# Autodesk Inventor assembly: 3D HUMAN
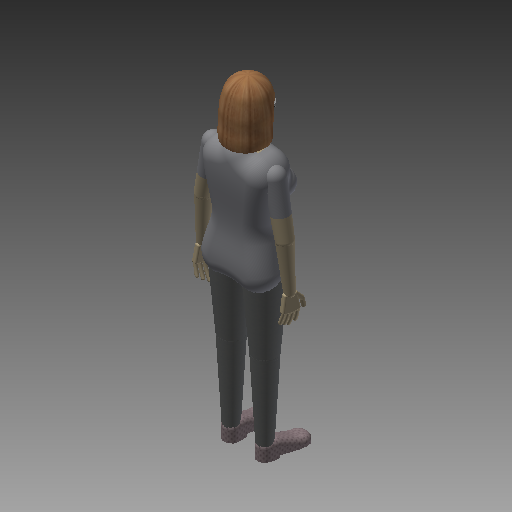
[picture p0: Inventor's stored thumbnail of the model, 512x512]
Saved by Autodesk Inventor 2019 (Build 230136000, 136)
## iProperties
Category: ASSY
Shininess: 64.0
Length Units: 11272
Angle Units: 11279
Time Units: 11290
Mass Units: 11286
Length Display Precision: 3
Angle Display Precision: 2
Compacted: True
Part Number: 3D HUMAN
Document SubType Name: Assembly
Created: 2003-03-22
Designer: M.F.
Catalog Web Link: www.apollocanard.com
Density: 0.0
Volumn: 0.0
Area: 0.0
PropertySet Name: Model Information
Control State: 0
Master: False
Checked Out: False
Title: iMandy
Author: M.F.
## Documents named in this file (14)
- \\Mac\Home\Downloads\iManikins\iMandy\iMandy.iam
- \\Mac\Home\Downloads\iManikins\iMandy\iMandy - 2D BODY.ipt
- \\Mac\Home\Downloads\iManikins\iMandy\iMandy - HAIR.ipt
- \\Mac\Home\Downloads\iManikins\iMandy\iMandy - HEAD.ipt
- \\Mac\Home\Downloads\iManikins\iMandy\iMandy - ARM UPPER.ipt
- \\Mac\Home\Downloads\iManikins\iMandy\iMandy - ARM LOWER.ipt
- \\Mac\Home\Downloads\iManikins\iMandy\iMandy - LEG UPPER.ipt
- \\Mac\Home\Downloads\iManikins\iMandy\iMandy - LEG LOWER.ipt
- \\Mac\Home\Downloads\iManikins\iMandy\iMandy - FOOT.ipt
- \\Mac\Home\Downloads\iManikins\iMandy\iMandy - HAND.ipt
- \\Mac\Home\Downloads\iManikins\iMandy\iMandy - FINGERS LEFT.ipt
- \\Mac\Home\Downloads\iManikins\iMandy\iMandy - FINGERS RIGHT.ipt
- \\Mac\Home\Downloads\iManikins\iMandy\iMandy - SHADES.ipt
- \\Mac\Home\Downloads\iManikins\iMandy\iMandy - TORSO.ipt
## Components (19 placed, 13 different names)
1. iMandy - 2D BODY:1 — Flush:1, Flush:2, Flush:7
2. iMandy - TORSO:1 — Flush:4, Flush:6, LEFT FOOT TWIST ANGLE, LEG STRADDLE DIST1, LEG STRADDLE DIST2, Flush:7, LEFT FOOT FLAT, RIGHT FOOT FLAT, Tangent:3, Mate:17
3. iMandy - ARM UPPER:1 — Mate:1
4. iMandy - ARM LOWER:1 — Mate:1, Mate:4
5. iMandy - LEG UPPER:1 — Mate:2
6. iMandy - LEG LOWER:1 — Mate:2, Mate:3, LEG STRADDLE DIST1, Tangent:1
7. iMandy - FOOT:1 — Mate:3, LEFT FOOT TWIST ANGLE, Tangent:1, LEFT FOOT FLAT
8. iMandy - HAND:1 — Mate:4, Mate:5, Mate:6, LEFT FINGERS CLOSED ANGLE
9. iMandy - FINGERS LEFT:1 — Mate:5, Mate:6, LEFT FINGERS CLOSED ANGLE
10. iMandy - ARM UPPER:2 — Mate:7
11. iMandy - ARM LOWER:2 — Mate:7, Mate:10, Mate:11
12. iMandy - LEG UPPER:2 — Mate:8
13. iMandy - LEG LOWER:2 — Mate:8, Mate:9, LEG STRADDLE DIST2, Tangent:2
14. iMandy - FOOT:2 — Mate:9, Tangent:2, RIGHT FOOT FLAT
15. iMandy - HAND:2 — Mate:10, Mate:11, Flush:3, Mate:12, RIGHT FINGERS CLOSED ANGLE
16. iMandy - FINGERS RIGHT:1 — Flush:3, Mate:12, RIGHT FINGERS CLOSED ANGLE
17. iMandy - SHADES:1 — Tangent:4, Angle:2, Mate:20
18. iMandy - HAIR:1 — Mate:21
19. iMandy - HEAD:1 — Tangent:3, Mate:17, Tangent:4, Angle:2, Mate:20, Mate:21
## Relationships (44: Mate 24, Flush 9, Angle 7, Tangent 4)
- Flush:1: iMandy - 2D BODY:1
- Flush:2: iMandy - 2D BODY:1
- Mate:1: iMandy - ARM UPPER:1 ↔ iMandy - ARM LOWER:1
- Mate:2: iMandy - LEG UPPER:1 ↔ iMandy - LEG LOWER:1
- Mate:3: iMandy - LEG LOWER:1 ↔ iMandy - FOOT:1
- Mate:4: iMandy - ARM LOWER:1 ↔ iMandy - HAND:1
- Mate:5: iMandy - HAND:1 ↔ iMandy - FINGERS LEFT:1
- Mate:6: iMandy - HAND:1 ↔ iMandy - FINGERS LEFT:1
- [Mate]: iMandy - ARM LOWER:1 ↔ iMandy - HAND:1
- LEFT FINGERS CLOSED ANGLE [Angle] (15 deg): iMandy - HAND:1 ↔ iMandy - FINGERS LEFT:1
- Mate:7: iMandy - ARM UPPER:2 ↔ iMandy - ARM LOWER:2
- Mate:8: iMandy - LEG UPPER:2 ↔ iMandy - LEG LOWER:2
- Mate:9: iMandy - LEG LOWER:2 ↔ iMandy - FOOT:2
- Mate:10: iMandy - ARM LOWER:2 ↔ iMandy - HAND:2
- Mate:11: iMandy - ARM LOWER:2 ↔ iMandy - HAND:2
- Flush:3: iMandy - HAND:2 ↔ iMandy - FINGERS RIGHT:1
- Mate:12: iMandy - HAND:2 ↔ iMandy - FINGERS RIGHT:1
- RIGHT FINGERS CLOSED ANGLE [Angle] (-15 deg): iMandy - HAND:2 ↔ iMandy - FINGERS RIGHT:1
- [Mate]: iMandy - TORSO:1 ↔ iMandy - ARM UPPER:1
- Flush:4: iMandy - TORSO:1
- [Flush]: iMandy - TORSO:1
- Flush:6: iMandy - TORSO:1
- LEFT FOOT TWIST ANGLE [Angle] (5 deg): iMandy - TORSO:1 ↔ iMandy - FOOT:1
- [Mate]: iMandy - TORSO:1 ↔ iMandy - ARM UPPER:2
- LEG STRADDLE DIST1 [Flush] (71.12 mm): iMandy - TORSO:1 ↔ iMandy - LEG LOWER:1
- LEG STRADDLE DIST2 [Flush] (-71.12 mm): iMandy - TORSO:1 ↔ iMandy - LEG LOWER:2
- [Angle] (5 deg): iMandy - TORSO:1 ↔ iMandy - FOOT:2
- Flush:7: iMandy - 2D BODY:1 ↔ iMandy - TORSO:1
- [Mate]: iMandy - TORSO:1 ↔ iMandy - LEG UPPER:1
- [Mate]: iMandy - TORSO:1 ↔ iMandy - LEG UPPER:2
- Tangent:1: iMandy - LEG LOWER:1 ↔ iMandy - FOOT:1
- Tangent:2: iMandy - LEG LOWER:2 ↔ iMandy - FOOT:2
- LEFT FOOT FLAT [Angle] (180 deg): iMandy - TORSO:1 ↔ iMandy - FOOT:1
- RIGHT FOOT FLAT [Angle] (-180 deg): iMandy - TORSO:1 ↔ iMandy - FOOT:2
- Tangent:3: iMandy - TORSO:1 ↔ iMandy - HEAD:1
- Mate:17: iMandy - TORSO:1 ↔ iMandy - HEAD:1
- [Mate] (19.05 mm): iMandy - TORSO:1 ↔ iMandy - HEAD:1
- [Mate]: iMandy - HAIR:1 ↔ iMandy - HEAD:1
- Tangent:4: iMandy - SHADES:1 ↔ iMandy - HEAD:1
- Angle:2 (3 deg): iMandy - SHADES:1 ↔ iMandy - HEAD:1
- Mate:20: iMandy - SHADES:1 ↔ iMandy - HEAD:1
- Mate:21: iMandy - HAIR:1 ↔ iMandy - HEAD:1
- [Mate]: iMandy - HAIR:1 ↔ iMandy - HEAD:1
- [Mate]: iMandy - SHADES:1 ↔ iMandy - HEAD:1
## Named parameters: LEG_STRADDLE_DIST_UNDER = 71.12 mm, LEFT_FINGERS_CLOSED_ANGLE = 15 deg, RIGHT_FINGERS_CLOSED_ANGLE = -15 deg
